# Autodesk Inventor assembly: FerriteCoreMem-1KB
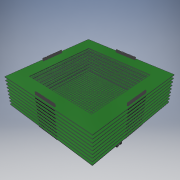
[picture p0: Inventor's stored thumbnail of the model, 180x180]
Saved by Autodesk Inventor 2018 (Build 220112000, 112)
## iProperties
Created: 2025-02-17
Part Number: FerriteCoreMem-1KB
Material: Všeobecné
Document SubType Name: Assembly
Designer: Jozko Mrkvicka
Author: Jozko Mrkvicka
## Documents named in this file (9)
- D:\05_Projekty\Projects_Inventor\Haluska9000\FerriteCoreMem-1KB.iam
- D:\05_Projekty\Projects_Inventor\Haluska9000\PinHeader-Female.ipt
- D:\05_Projekty\Projects_Inventor\Haluska9000\PCB-FerriteCore\PCB-FerriteCore#HighPoly.ipt
- D:\05_Projekty\Projects_Inventor\Haluska9000\PCB-FerriteCore.ipt
- D:\05_Projekty\Projects_Inventor\Haluska9000\PCB-FerriteCore\PCB-FerriteCore#LowPoly.ipt
- D:\05_Projekty\Projects_Inventor\Haluska9000\FerriteCoreMesh.ipt
- D:\05_Projekty\Projects_Inventor\Haluska9000\PinHeader-Female(LowPoly).ipt
- D:\05_Projekty\Projects_Inventor\Haluska9000\PCB-FerriteCore\PCB-FerriteCore#Decoder.ipt
- D:\05_Projekty\Common\Library_Inventor\PinHeader-2x5-Male-Bent.ipt
## Components (47 placed, 7 different names)
1. PCB-FerriteCore#HighPoly:1 — Stejný směr:35, Stejný směr:36, Proti sobě:466, Proti sobě:467, Proti sobě:468, Proti sobě:469, Proti sobě:470, Proti sobě:471, Proti sobě:472, Proti sobě:473, Proti sobě:474, Proti sobě:475, Stejný směr:101
2. FerriteCoreMesh:1 — Stejný směr:35, Stejný směr:36, Stejný směr:101
3. PinHeader-Female:1 — Proti sobě:466, Stejný směr:102, Stejný směr:103
4. PinHeader-Female(LowPoly):1 — Stejný směr:37, Proti sobě:476, Proti sobě:477, Stejný směr:38, Stejný směr:95, Stejný směr:96, Proti sobě:528
5. PinHeader-Female:2 — Proti sobě:467, Proti sobě:468, Proti sobě:469, Stejný směr:99, Stejný směr:100, Proti sobě:532
6. PinHeader-Female:3 — Proti sobě:470, Proti sobě:471, Proti sobě:472
7. PinHeader-Female:4 — Proti sobě:473, Proti sobě:474, Proti sobě:475
8. PCB-FerriteCore#LowPoly:2 — Stejný směr:37, Proti sobě:476, Proti sobě:477, Proti sobě:479, Stejný směr:39, Stejný směr:40, Proti sobě:480, Proti sobě:481, Stejný směr:42, Proti sobě:482, Proti sobě:527
9. PinHeader-Female(LowPoly):2 — Stejný směr:38, Proti sobě:479, Stejný směr:39
10. PinHeader-Female(LowPoly):3 — Stejný směr:40, Proti sobě:480, Proti sobě:481, Stejný směr:41, Stejný směr:87, Stejný směr:88
11. PinHeader-Female(LowPoly):4 — Stejný směr:41, Stejný směr:42, Proti sobě:482
12. PinHeader-Female(LowPoly):5 — Stejný směr:96, Stejný směr:97, Proti sobě:527
13. PCB-FerriteCore#LowPoly:3 — Proti sobě:526
14. PinHeader-Female(LowPoly):6
15. PinHeader-Female(LowPoly):7 — Stejný směr:86, Stejný směr:87
16. PinHeader-Female(LowPoly):8
17. PinHeader-Female(LowPoly):9 — Stejný směr:94, Stejný směr:95, Proti sobě:529
18. PCB-FerriteCore#LowPoly:4 — Proti sobě:528
19. PinHeader-Female(LowPoly):10
20. PinHeader-Female(LowPoly):11 — Stejný směr:88, Stejný směr:89
21. PinHeader-Female(LowPoly):12
22. PinHeader-Female(LowPoly):13 — Stejný směr:93, Stejný směr:94, Proti sobě:530
23. PCB-FerriteCore#LowPoly:5 — Proti sobě:529
24. PinHeader-Female(LowPoly):14
25. PinHeader-Female(LowPoly):15 — Stejný směr:89, Stejný směr:90
26. PinHeader-Female(LowPoly):16
27. PinHeader-Female(LowPoly):17 — Stejný směr:93, Stejný směr:113, Proti sobě:538
28. PCB-FerriteCore#LowPoly:6 — Proti sobě:530, Stejný směr:104, Stejný směr:105
29. PinHeader-Female(LowPoly):18 — Proti sobě:533, Stejný směr:110, Stejný směr:111, Proti sobě:535
30. PinHeader-Female(LowPoly):19 — Stejný směr:90, Proti sobě:537, Stejný směr:112
31. PinHeader-Female(LowPoly):20 — Stejný směr:108, Stejný směr:109, Proti sobě:534
32. PinHeader-Female(LowPoly):25 — Stejný směr:97, Stejný směr:98, Proti sobě:526
33. PCB-FerriteCore#LowPoly:8 — Proti sobě:525
34. PinHeader-Female(LowPoly):26
35. PinHeader-Female(LowPoly):27 — Stejný směr:85, Stejný směr:86
36. PinHeader-Female(LowPoly):28
37. PinHeader-Female(LowPoly):29 — Stejný směr:98, Proti sobě:525, Stejný směr:99, Stejný směr:100
38. PCB-FerriteCore#LowPoly:9 — Proti sobě:532
39. PinHeader-Female(LowPoly):30 — Stejný směr:102, Stejný směr:103
40. PinHeader-Female(LowPoly):31 — Stejný směr:85
41. PinHeader-Female(LowPoly):32
42. PCB-FerriteCore#Decoder:10 — Stejný směr:104, Stejný směr:105, Proti sobě:533, Proti sobě:539, Proti sobě:540, Proti sobě:541
43. PinHeader-Female(LowPoly):33 — Stejný směr:113, Proti sobě:538
44. PinHeader-Female(LowPoly):34 — Stejný směr:110, Stejný směr:111, Proti sobě:535
45. PinHeader-Female(LowPoly):35 — Proti sobě:537, Stejný směr:112
46. PinHeader-Female(LowPoly):36 — Stejný směr:108, Stejný směr:109, Proti sobě:534
47. PinHeader-2x5-Male-Bent:1 — Proti sobě:539, Proti sobě:540, Proti sobě:541
## Relationships (138: Flush 71, Mate 67)
- Stejný směr:35 [Flush]: PCB-FerriteCore#HighPoly:1 ↔ FerriteCoreMesh:1
- Stejný směr:36 [Flush]: PCB-FerriteCore#HighPoly:1 ↔ FerriteCoreMesh:1
- Proti sobě:466 [Mate]: PCB-FerriteCore#HighPoly:1 ↔ PinHeader-Female:1
- Proti sobě:467 [Mate]: PCB-FerriteCore#HighPoly:1 ↔ PinHeader-Female:2
- Proti sobě:468 [Mate]: PCB-FerriteCore#HighPoly:1 ↔ PinHeader-Female:2
- Proti sobě:469 [Mate]: PCB-FerriteCore#HighPoly:1 ↔ PinHeader-Female:2
- Proti sobě:470 [Mate]: PCB-FerriteCore#HighPoly:1 ↔ PinHeader-Female:3
- Proti sobě:471 [Mate]: PCB-FerriteCore#HighPoly:1 ↔ PinHeader-Female:3
- Proti sobě:472 [Mate]: PCB-FerriteCore#HighPoly:1 ↔ PinHeader-Female:3
- Proti sobě:473 [Mate]: PCB-FerriteCore#HighPoly:1 ↔ PinHeader-Female:4
- Proti sobě:474 [Mate]: PCB-FerriteCore#HighPoly:1 ↔ PinHeader-Female:4
- Proti sobě:475 [Mate]: PCB-FerriteCore#HighPoly:1 ↔ PinHeader-Female:4
- Stejný směr:37 [Flush]: PinHeader-Female(LowPoly):1 ↔ PCB-FerriteCore#LowPoly:2
- Proti sobě:476 [Mate]: PinHeader-Female(LowPoly):1 ↔ PCB-FerriteCore#LowPoly:2
- Proti sobě:477 [Mate]: PinHeader-Female(LowPoly):1 ↔ PCB-FerriteCore#LowPoly:2
- Stejný směr:38 [Flush]: PinHeader-Female(LowPoly):1 ↔ PinHeader-Female(LowPoly):2
- Proti sobě:479 [Mate]: PCB-FerriteCore#LowPoly:2 ↔ PinHeader-Female(LowPoly):2
- Stejný směr:39 [Flush]: PCB-FerriteCore#LowPoly:2 ↔ PinHeader-Female(LowPoly):2
- Stejný směr:40 [Flush]: PCB-FerriteCore#LowPoly:2 ↔ PinHeader-Female(LowPoly):3
- Proti sobě:480 [Mate]: PCB-FerriteCore#LowPoly:2 ↔ PinHeader-Female(LowPoly):3
- Proti sobě:481 [Mate]: PCB-FerriteCore#LowPoly:2 ↔ PinHeader-Female(LowPoly):3
- Stejný směr:41 [Flush]: PinHeader-Female(LowPoly):3 ↔ PinHeader-Female(LowPoly):4
- Stejný směr:42 [Flush]: PCB-FerriteCore#LowPoly:2 ↔ PinHeader-Female(LowPoly):4
- Proti sobě:482 [Mate]: PCB-FerriteCore#LowPoly:2 ↔ PinHeader-Female(LowPoly):4
- [Flush]: PinHeader-Female(LowPoly):5 ↔ PCB-FerriteCore#LowPoly:3
- [Mate]: PinHeader-Female(LowPoly):5 ↔ PCB-FerriteCore#LowPoly:3
- [Mate]: PinHeader-Female(LowPoly):5 ↔ PCB-FerriteCore#LowPoly:3
- [Flush]: PinHeader-Female(LowPoly):5 ↔ PinHeader-Female(LowPoly):6
- [Mate]: PCB-FerriteCore#LowPoly:3 ↔ PinHeader-Female(LowPoly):6
- [Flush]: PCB-FerriteCore#LowPoly:3 ↔ PinHeader-Female(LowPoly):6
- [Flush]: PCB-FerriteCore#LowPoly:3 ↔ PinHeader-Female(LowPoly):7
- [Mate]: PCB-FerriteCore#LowPoly:3 ↔ PinHeader-Female(LowPoly):7
- [Mate]: PCB-FerriteCore#LowPoly:3 ↔ PinHeader-Female(LowPoly):7
- [Flush]: PinHeader-Female(LowPoly):7 ↔ PinHeader-Female(LowPoly):8
- [Flush]: PCB-FerriteCore#LowPoly:3 ↔ PinHeader-Female(LowPoly):8
- [Mate]: PCB-FerriteCore#LowPoly:3 ↔ PinHeader-Female(LowPoly):8
- [Flush]: PinHeader-Female(LowPoly):9 ↔ PCB-FerriteCore#LowPoly:4
- [Mate]: PinHeader-Female(LowPoly):9 ↔ PCB-FerriteCore#LowPoly:4
- [Mate]: PinHeader-Female(LowPoly):9 ↔ PCB-FerriteCore#LowPoly:4
- [Flush]: PinHeader-Female(LowPoly):9 ↔ PinHeader-Female(LowPoly):10
- [Mate]: PCB-FerriteCore#LowPoly:4 ↔ PinHeader-Female(LowPoly):10
- [Flush]: PCB-FerriteCore#LowPoly:4 ↔ PinHeader-Female(LowPoly):10
- [Flush]: PCB-FerriteCore#LowPoly:4 ↔ PinHeader-Female(LowPoly):11
- [Mate]: PCB-FerriteCore#LowPoly:4 ↔ PinHeader-Female(LowPoly):11
- [Mate]: PCB-FerriteCore#LowPoly:4 ↔ PinHeader-Female(LowPoly):11
- [Flush]: PinHeader-Female(LowPoly):11 ↔ PinHeader-Female(LowPoly):12
- [Flush]: PCB-FerriteCore#LowPoly:4 ↔ PinHeader-Female(LowPoly):12
- [Mate]: PCB-FerriteCore#LowPoly:4 ↔ PinHeader-Female(LowPoly):12
- [Flush]: PinHeader-Female(LowPoly):13 ↔ PCB-FerriteCore#LowPoly:5
- [Mate]: PinHeader-Female(LowPoly):13 ↔ PCB-FerriteCore#LowPoly:5
- [Mate]: PinHeader-Female(LowPoly):13 ↔ PCB-FerriteCore#LowPoly:5
- [Flush]: PinHeader-Female(LowPoly):13 ↔ PinHeader-Female(LowPoly):14
- [Mate]: PCB-FerriteCore#LowPoly:5 ↔ PinHeader-Female(LowPoly):14
- [Flush]: PCB-FerriteCore#LowPoly:5 ↔ PinHeader-Female(LowPoly):14
- [Flush]: PCB-FerriteCore#LowPoly:5 ↔ PinHeader-Female(LowPoly):15
- [Mate]: PCB-FerriteCore#LowPoly:5 ↔ PinHeader-Female(LowPoly):15
- [Mate]: PCB-FerriteCore#LowPoly:5 ↔ PinHeader-Female(LowPoly):15
- [Flush]: PinHeader-Female(LowPoly):15 ↔ PinHeader-Female(LowPoly):16
- [Flush]: PCB-FerriteCore#LowPoly:5 ↔ PinHeader-Female(LowPoly):16
- [Mate]: PCB-FerriteCore#LowPoly:5 ↔ PinHeader-Female(LowPoly):16
- [Flush]: PinHeader-Female(LowPoly):17 ↔ PCB-FerriteCore#LowPoly:6
- [Mate]: PinHeader-Female(LowPoly):17 ↔ PCB-FerriteCore#LowPoly:6
- [Mate]: PinHeader-Female(LowPoly):17 ↔ PCB-FerriteCore#LowPoly:6
- [Flush]: PinHeader-Female(LowPoly):17 ↔ PinHeader-Female(LowPoly):18
- [Mate]: PCB-FerriteCore#LowPoly:6 ↔ PinHeader-Female(LowPoly):18
- [Flush]: PCB-FerriteCore#LowPoly:6 ↔ PinHeader-Female(LowPoly):18
- [Flush]: PCB-FerriteCore#LowPoly:6 ↔ PinHeader-Female(LowPoly):19
- [Mate]: PCB-FerriteCore#LowPoly:6 ↔ PinHeader-Female(LowPoly):19
- [Mate]: PCB-FerriteCore#LowPoly:6 ↔ PinHeader-Female(LowPoly):19
- [Flush]: PinHeader-Female(LowPoly):19 ↔ PinHeader-Female(LowPoly):20
- [Flush]: PCB-FerriteCore#LowPoly:6 ↔ PinHeader-Female(LowPoly):20
- [Mate]: PCB-FerriteCore#LowPoly:6 ↔ PinHeader-Female(LowPoly):20
- [Flush]: PinHeader-Female(LowPoly):25 ↔ PCB-FerriteCore#LowPoly:8
- [Mate]: PinHeader-Female(LowPoly):25 ↔ PCB-FerriteCore#LowPoly:8
- [Mate]: PinHeader-Female(LowPoly):25 ↔ PCB-FerriteCore#LowPoly:8
- [Flush]: PinHeader-Female(LowPoly):25 ↔ PinHeader-Female(LowPoly):26
- [Mate]: PCB-FerriteCore#LowPoly:8 ↔ PinHeader-Female(LowPoly):26
- [Flush]: PCB-FerriteCore#LowPoly:8 ↔ PinHeader-Female(LowPoly):26
- [Flush]: PCB-FerriteCore#LowPoly:8 ↔ PinHeader-Female(LowPoly):27
- [Mate]: PCB-FerriteCore#LowPoly:8 ↔ PinHeader-Female(LowPoly):27
- [Mate]: PCB-FerriteCore#LowPoly:8 ↔ PinHeader-Female(LowPoly):27
- [Flush]: PinHeader-Female(LowPoly):27 ↔ PinHeader-Female(LowPoly):28
- [Flush]: PCB-FerriteCore#LowPoly:8 ↔ PinHeader-Female(LowPoly):28
- [Mate]: PCB-FerriteCore#LowPoly:8 ↔ PinHeader-Female(LowPoly):28
- [Flush]: PinHeader-Female(LowPoly):29 ↔ PCB-FerriteCore#LowPoly:9
- [Mate]: PinHeader-Female(LowPoly):29 ↔ PCB-FerriteCore#LowPoly:9
- [Mate]: PinHeader-Female(LowPoly):29 ↔ PCB-FerriteCore#LowPoly:9
- [Flush]: PinHeader-Female(LowPoly):29 ↔ PinHeader-Female(LowPoly):30
- [Mate]: PCB-FerriteCore#LowPoly:9 ↔ PinHeader-Female(LowPoly):30
- [Flush]: PCB-FerriteCore#LowPoly:9 ↔ PinHeader-Female(LowPoly):30
- [Flush]: PCB-FerriteCore#LowPoly:9 ↔ PinHeader-Female(LowPoly):31
- [Mate]: PCB-FerriteCore#LowPoly:9 ↔ PinHeader-Female(LowPoly):31
- [Mate]: PCB-FerriteCore#LowPoly:9 ↔ PinHeader-Female(LowPoly):31
- [Flush]: PinHeader-Female(LowPoly):31 ↔ PinHeader-Female(LowPoly):32
- [Flush]: PCB-FerriteCore#LowPoly:9 ↔ PinHeader-Female(LowPoly):32
- [Mate]: PCB-FerriteCore#LowPoly:9 ↔ PinHeader-Female(LowPoly):32
- Stejný směr:85 [Flush]: PinHeader-Female(LowPoly):27 ↔ PinHeader-Female(LowPoly):31
- Stejný směr:86 [Flush]: PinHeader-Female(LowPoly):7 ↔ PinHeader-Female(LowPoly):27
- Stejný směr:87 [Flush]: PinHeader-Female(LowPoly):3 ↔ PinHeader-Female(LowPoly):7
- Stejný směr:88 [Flush]: PinHeader-Female(LowPoly):3 ↔ PinHeader-Female(LowPoly):11
- Stejný směr:89 [Flush]: PinHeader-Female(LowPoly):11 ↔ PinHeader-Female(LowPoly):15
- Stejný směr:90 [Flush]: PinHeader-Female(LowPoly):15 ↔ PinHeader-Female(LowPoly):19
- Stejný směr:93 [Flush]: PinHeader-Female(LowPoly):13 ↔ PinHeader-Female(LowPoly):17
- Stejný směr:94 [Flush]: PinHeader-Female(LowPoly):9 ↔ PinHeader-Female(LowPoly):13
- Stejný směr:95 [Flush]: PinHeader-Female(LowPoly):1 ↔ PinHeader-Female(LowPoly):9
- Stejný směr:96 [Flush]: PinHeader-Female(LowPoly):1 ↔ PinHeader-Female(LowPoly):5
- Stejný směr:97 [Flush]: PinHeader-Female(LowPoly):5 ↔ PinHeader-Female(LowPoly):25
- Stejný směr:98 [Flush]: PinHeader-Female(LowPoly):25 ↔ PinHeader-Female(LowPoly):29
- Proti sobě:525 [Mate]: PCB-FerriteCore#LowPoly:8 ↔ PinHeader-Female(LowPoly):29
- Proti sobě:526 [Mate]: PCB-FerriteCore#LowPoly:3 ↔ PinHeader-Female(LowPoly):25
- Proti sobě:527 [Mate]: PCB-FerriteCore#LowPoly:2 ↔ PinHeader-Female(LowPoly):5
- Proti sobě:528 [Mate]: PinHeader-Female(LowPoly):1 ↔ PCB-FerriteCore#LowPoly:4
- Proti sobě:529 [Mate]: PinHeader-Female(LowPoly):9 ↔ PCB-FerriteCore#LowPoly:5
- Proti sobě:530 [Mate]: PinHeader-Female(LowPoly):13 ↔ PCB-FerriteCore#LowPoly:6
- Stejný směr:99 [Flush]: PinHeader-Female:2 ↔ PinHeader-Female(LowPoly):29
- Stejný směr:100 [Flush]: PinHeader-Female:2 ↔ PinHeader-Female(LowPoly):29
- Proti sobě:532 [Mate]: PinHeader-Female:2 ↔ PCB-FerriteCore#LowPoly:9
- Stejný směr:101 [Flush]: PCB-FerriteCore#HighPoly:1 ↔ FerriteCoreMesh:1
- Stejný směr:102 [Flush]: PinHeader-Female:1 ↔ PinHeader-Female(LowPoly):30
- Stejný směr:103 [Flush]: PinHeader-Female:1 ↔ PinHeader-Female(LowPoly):30
- Stejný směr:104 [Flush]: PCB-FerriteCore#LowPoly:6 ↔ PCB-FerriteCore#Decoder:10
- Stejný směr:105 [Flush]: PCB-FerriteCore#LowPoly:6 ↔ PCB-FerriteCore#Decoder:10
- Proti sobě:533 [Mate]: PinHeader-Female(LowPoly):18 ↔ PCB-FerriteCore#Decoder:10
- [Flush]: PinHeader-Female(LowPoly):33 ↔ PinHeader-Female(LowPoly):34
- [Flush]: PinHeader-Female(LowPoly):35 ↔ PinHeader-Female(LowPoly):36
- Stejný směr:108 [Flush]: PinHeader-Female(LowPoly):20 ↔ PinHeader-Female(LowPoly):36
- Stejný směr:109 [Flush]: PinHeader-Female(LowPoly):20 ↔ PinHeader-Female(LowPoly):36
- Proti sobě:534 [Mate]: PinHeader-Female(LowPoly):20 ↔ PinHeader-Female(LowPoly):36
- Stejný směr:110 [Flush]: PinHeader-Female(LowPoly):18 ↔ PinHeader-Female(LowPoly):34
- Stejný směr:111 [Flush]: PinHeader-Female(LowPoly):18 ↔ PinHeader-Female(LowPoly):34
- Proti sobě:535 [Mate]: PinHeader-Female(LowPoly):18 ↔ PinHeader-Female(LowPoly):34
- Proti sobě:537 [Mate]: PinHeader-Female(LowPoly):19 ↔ PinHeader-Female(LowPoly):35
- Stejný směr:112 [Flush]: PinHeader-Female(LowPoly):19 ↔ PinHeader-Female(LowPoly):35
- Stejný směr:113 [Flush]: PinHeader-Female(LowPoly):17 ↔ PinHeader-Female(LowPoly):33
- Proti sobě:538 [Mate]: PinHeader-Female(LowPoly):17 ↔ PinHeader-Female(LowPoly):33
- Proti sobě:539 [Mate]: PCB-FerriteCore#Decoder:10 ↔ PinHeader-2x5-Male-Bent:1
- Proti sobě:540 [Mate]: PCB-FerriteCore#Decoder:10 ↔ PinHeader-2x5-Male-Bent:1
- Proti sobě:541 [Mate]: PCB-FerriteCore#Decoder:10 ↔ PinHeader-2x5-Male-Bent:1
## Named parameters: d743_d729 = 0 mm, d744_d731 = 0 mm, d745_d732 = 0 mm, d746_d733 = 0 mm, d747_d735 = 0 mm, d748_d736 = 0 mm, d749_d737 = 0 mm, d750_d738 = 0 mm, d751_d739 = 0 mm, d752_d740 = 0 mm, d753_d741 = 0 mm, d754_d742 = 0 mm, d755_d729 = 0 mm, d756_d731 = 0 mm, d757_d732 = 0 mm, d758_d733 = 0 mm, d759_d735 = 0 mm, d760_d736 = 0 mm, d761_d737 = 0 mm, d762_d738 = 0 mm, d763_d739 = 0 mm, d764_d740 = 0 mm, d765_d741 = 0 mm, d766_d742 = 0 mm, d767_d729 = 0 mm, d768_d731 = 0 mm, d769_d732 = 0 mm, d770_d733 = 0 mm, d771_d735 = 0 mm, d772_d736 = 0 mm, d773_d737 = 0 mm, d774_d738 = 0 mm, d775_d739 = 0 mm, d776_d740 = 0 mm, d777_d741 = 0 mm, d778_d742 = 0 mm, d779_d729 = 0 mm, d780_d731 = 0 mm, d781_d732 = 0 mm, d782_d733 = 0 mm, d783_d735 = 0 mm, d784_d736 = 0 mm, d785_d737 = 0 mm, d786_d738 = 0 mm, d787_d739 = 0 mm, d788_d740 = 0 mm, d789_d741 = 0 mm, d790_d742 = 0 mm, d803_d729 = 0 mm, d804_d731 = 0 mm, d805_d732 = 0 mm, d806_d733 = 0 mm, d807_d735 = 0 mm, d808_d736 = 0 mm, d809_d737 = 0 mm, d810_d738 = 0 mm, d811_d739 = 0 mm, d812_d740 = 0 mm, d813_d741 = 0 mm, d814_d742 = 0 mm, d815_d729 = 0 mm, d816_d731 = 0 mm, d817_d732 = 0 mm, d818_d733 = 0 mm, d819_d735 = 0 mm, d820_d736 = 0 mm, d821_d737 = 0 mm, d822_d738 = 0 mm, d823_d739 = 0 mm, d824_d740 = 0 mm, d825_d741 = 0 mm, d826_d742 = 0 mm, d857_d782_d733 = 0 mm, d858_d788_d740 = 0 mm
